# Autodesk Inventor assembly: ASM_HDR50_Motor_and_ConnectorPlate
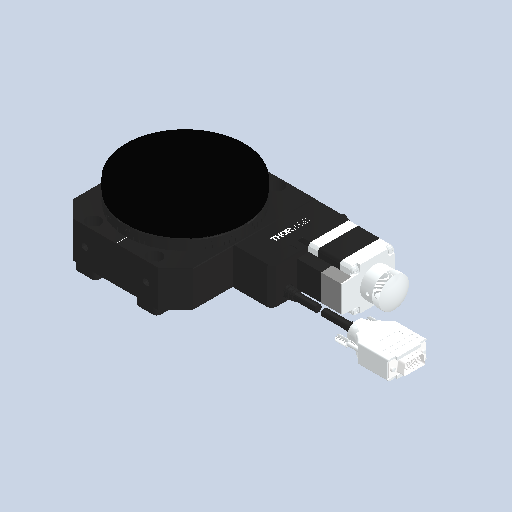
[picture p0: Inventor's stored thumbnail of the model, 512x512]
Saved by Autodesk Inventor 2024 (Build 280153000, 153)
## iProperties
Created: 2024-03-28
Part Number: ASM_HDR50_Motor_and_ConnectorPlate
Document SubType Name: Assembly
Designer: jamha
Author: jamha
## Documents named in this file (3)
- C:\Users\jamha\OneDrive - The University of Texas at Dallas\SD - TEAM 1830\CAD\James\CAD Final Deliverable\ASM_HDR50_Motor_and_ConnectorPlate.iam
- C:\Users\jamha\OneDrive - The University of Texas at Dallas\SD - TEAM 1830\CAD\James\CAD Final Deliverable\IPT_HDR50_Stepper_Motor.ipt
- C:\Users\jamha\OneDrive - The University of Texas at Dallas\SD - TEAM 1830\CAD\James\CAD Final Deliverable\IPT_Adapter_Plate.ipt
## Components (2 placed, 2 different names)
1. HDR50-Step:1 — Mate:1, Mate:2, Mate:3
2. NR360SP9_M-Step:1 — Mate:1, Mate:2, Mate:3
## Relationships (3: Mate 3)
- Mate:1: HDR50-Step:1 ↔ NR360SP9_M-Step:1
- Mate:2: HDR50-Step:1 ↔ NR360SP9_M-Step:1
- Mate:3: HDR50-Step:1 ↔ NR360SP9_M-Step:1
